# Autodesk Inventor assembly: Roller Carouel Assembly
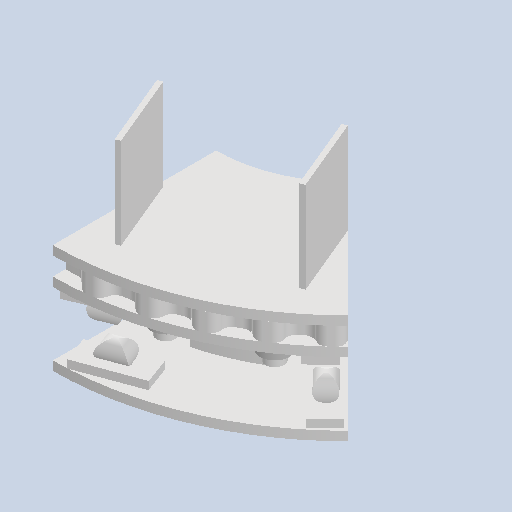
[picture p0: Inventor's stored thumbnail of the model, 512x512]
Saved by Autodesk Inventor 2023 (Build 270158000, 158)
## iProperties
Created: 2022-11-09
Part Number: Roller Carouel Assembly
Document SubType Name: Assembly
Designer: cheng
Author: cheng
## Documents named in this file (6)
- C:\Users\cheng\Desktop\4th Year Project\Inventor\Second Assembly\Second Assembly\Roller Carouel Assembly.iam
- C:\Users\cheng\Desktop\4th Year Project\Inventor\Second Assembly\Second Assembly\Roller Carousel Part.ipt
- C:\Users\cheng\Desktop\4th Year Project\Inventor\Second Assembly\Second Assembly\ball transfer unit.ipt
- C:\Users\cheng\Desktop\4th Year Project\Inventor\Second Assembly\Second Assembly\6002-z-bnl v1.ipt
- C:\Users\cheng\Desktop\4th Year Project\Inventor\Second Assembly\Second Assembly\Carousel Container Plate.ipt
- C:\Users\cheng\Desktop\4th Year Project\Inventor\Second Assembly\Second Assembly\Roller Carousel Gear.ipt
## Components (13 placed, 5 different names)
1. Roller Carousel Part:1 — Mate:1, Mate:2, Mate:3, Mate:4, Mate:5, Mate:6, Rotational:1, Rotational:2, Rotational:3, Rotational:4, Mate:7, Mate:8, Mate:9
2. ball transfer unit:1 — Mate:1
3. ball transfer unit:2 — Mate:2
4. ball transfer unit:4 — Mate:3
5. ball transfer unit:5 — Mate:4
6. ball transfer unit:6 — Mate:5
7. ball transfer unit:7 — Mate:6
8. 6002-z-bnl v1:1 — Rotational:3
9. 6002-z-bnl v1:2 — Rotational:1
10. 6002-z-bnl v1:3 — Rotational:4
11. 6002-z-bnl v1:4 — Rotational:2
12. Carousel Container Plate:1 — Mate:10, Mate:11, Mate:12
13. Roller Carousel Gear:1 — Mate:7, Mate:8, Mate:9, Mate:10, Mate:11, Mate:12
## Relationships (16: Mate 12, RevoluteJoint 4)
- Mate:1: Roller Carousel Part:1 ↔ ball transfer unit:1
- Mate:2: Roller Carousel Part:1 ↔ ball transfer unit:2
- Mate:3: Roller Carousel Part:1 ↔ ball transfer unit:4
- Mate:4: Roller Carousel Part:1 ↔ ball transfer unit:5
- Mate:5: Roller Carousel Part:1 ↔ ball transfer unit:6
- Mate:6: Roller Carousel Part:1 ↔ ball transfer unit:7
- Rotational:1 [RevoluteJoint]: Roller Carousel Part:1 ↔ 6002-z-bnl v1:2
- Rotational:2 [RevoluteJoint]: Roller Carousel Part:1 ↔ 6002-z-bnl v1:4
- Rotational:3 [RevoluteJoint]: Roller Carousel Part:1 ↔ 6002-z-bnl v1:1
- Rotational:4 [RevoluteJoint]: Roller Carousel Part:1 ↔ 6002-z-bnl v1:3
- Mate:7: Roller Carousel Part:1 ↔ Roller Carousel Gear:1
- Mate:8: Roller Carousel Part:1 ↔ Roller Carousel Gear:1
- Mate:9: Roller Carousel Part:1 ↔ Roller Carousel Gear:1
- Mate:10: Carousel Container Plate:1 ↔ Roller Carousel Gear:1
- Mate:11: Carousel Container Plate:1 ↔ Roller Carousel Gear:1
- Mate:12: Carousel Container Plate:1 ↔ Roller Carousel Gear:1
